# Autodesk Inventor assembly: kinect bracket
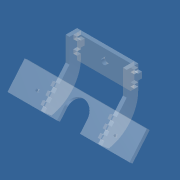
[picture p0: Inventor's stored thumbnail of the model, 180x180]
Saved by Autodesk Inventor 2012 (Build 160160000, 160)
## iProperties
Created: 2012-11-01
Part Number: kinect bracket
Document SubType Name: Assembly
Designer: Ed
Author: Ed
## Documents named in this file (4)
- C:\Users\Ed\Documents\masters\CAD\Kinect\acrylic kinect bracket.iam
- C:\Users\Ed\Documents\masters\CAD\Kinect\acrylic kinect bracket - bracket.ipt
- C:\Users\Ed\Documents\masters\CAD\Kinect\acrylic kinect plate.ipt
- C:\Users\Ed\Documents\masters\CAD\Kinect\acrylic kinect bracket - kinect plate.ipt
## Components (4 placed, 3 different names)
1. acrylic kinect bracket - bracket:1 — Mate:1, Mate:2, Mate:3
2. acrylic kinect bracket - bracket:2 — Mate:4, Mate:5, Mate:6, Mate:7, Mate:8, Mate:9
3. acrylic kinect plate:1 — Mate:1, Mate:2, Mate:3, Mate:4, Mate:5, Mate:6
4. acrylic kinect bracket - kinect plate:1 — Mate:7, Mate:8, Mate:9
## Relationships (9: Mate 9)
- Mate:1: acrylic kinect bracket - bracket:1 ↔ acrylic kinect plate:1
- Mate:2: acrylic kinect bracket - bracket:1 ↔ acrylic kinect plate:1
- Mate:3: acrylic kinect bracket - bracket:1 ↔ acrylic kinect plate:1
- Mate:4: acrylic kinect bracket - bracket:2 ↔ acrylic kinect plate:1
- Mate:5: acrylic kinect bracket - bracket:2 ↔ acrylic kinect plate:1
- Mate:6: acrylic kinect bracket - bracket:2 ↔ acrylic kinect plate:1
- Mate:7: acrylic kinect bracket - bracket:2 ↔ acrylic kinect bracket - kinect plate:1
- Mate:8: acrylic kinect bracket - bracket:2 ↔ acrylic kinect bracket - kinect plate:1
- Mate:9: acrylic kinect bracket - bracket:2 ↔ acrylic kinect bracket - kinect plate:1
